# Autodesk Inventor assembly: Suporte Inferior
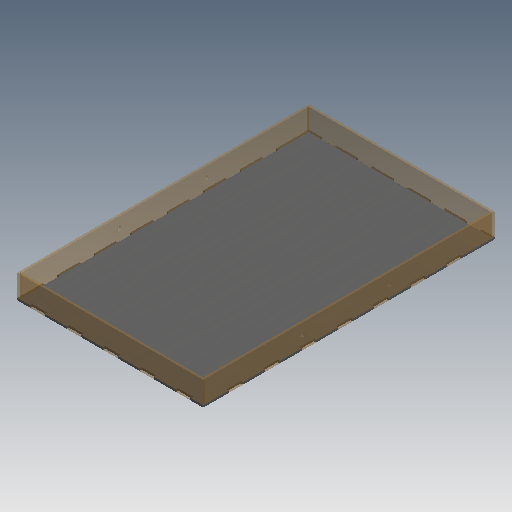
[picture p0: Inventor's stored thumbnail of the model, 512x512]
Saved by Autodesk Inventor 2020 (Build 240168000, 168)
## iProperties
Created: 2021-09-22
Part Number: Suporte Inferior
Document SubType Name: Assembly
Designer: pablo
Author: pablo
## Documents named in this file (4)
- C:\Google Drive\Pablo Arquivos\Projetos\Utilidades Domesticas\Talheres\Suporte Inferior.iam
- C:\Google Drive\Pablo Arquivos\Projetos\Utilidades Domesticas\Talheres\base inferior.ipt
- C:\Google Drive\Pablo Arquivos\Projetos\Utilidades Domesticas\Talheres\Divisória-30cm c rolamento - inferior.ipt
- C:\Google Drive\Pablo Arquivos\Projetos\Utilidades Domesticas\Talheres\Divisória-25cm.ipt
## Components (5 placed, 3 different names)
1. base inferior:1 — Mate:1, Mate:2, Mate:7, Mate:8, Mate:9, Mate:10, Mate:11, Mate:12
2. Divisória-30cm c rolamento - inferior:1 — Mate:9, Mate:10
3. Divisória-30cm c rolamento - inferior:2 — Mate:11, Mate:12
4. Divisória-25cm:1 — Mate:1, Mate:2
5. Divisória-25cm:2 — Mate:7, Mate:8
## Relationships (8: Mate 8)
- Mate:1: base inferior:1 ↔ Divisória-25cm:1
- Mate:2: base inferior:1 ↔ Divisória-25cm:1
- Mate:7: base inferior:1 ↔ Divisória-25cm:2
- Mate:8: base inferior:1 ↔ Divisória-25cm:2
- Mate:9: base inferior:1 ↔ Divisória-30cm c rolamento - inferior:1
- Mate:10: base inferior:1 ↔ Divisória-30cm c rolamento - inferior:1
- Mate:11: base inferior:1 ↔ Divisória-30cm c rolamento - inferior:2
- Mate:12: base inferior:1 ↔ Divisória-30cm c rolamento - inferior:2
